# Autodesk Inventor assembly: SpMax_steer
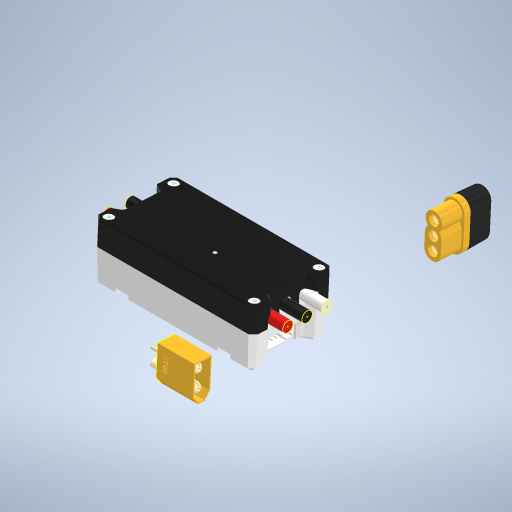
[picture p0: Inventor's stored thumbnail of the model, 512x512]
Saved by Autodesk Inventor 2023 (Build 270158000, 158)
## iProperties
Created: 2023-09-18
Part Number: SpMax_steer
Document SubType Name: Assembly
Designer: shpctac10011
Author: shpctac10011
## Documents named in this file (4)
- G:\.shortcut-targets-by-id\104lhnwPhYvankLacu8RGROV89Bx_24Mg\1939\2_Design\2023-2024\Parts\Electronics\SpMax_steer.iam
- G:\.shortcut-targets-by-id\104lhnwPhYvankLacu8RGROV89Bx_24Mg\1939\2_Design\2023-2024\Parts\Electronics\REV-11-2158-Spark-MAX_Wired.ipt
- G:\.shortcut-targets-by-id\104lhnwPhYvankLacu8RGROV89Bx_24Mg\1939\2_Design\2023-2024\Parts\Electronics\Connectors\XT60_Recp.ipt
- G:\.shortcut-targets-by-id\104lhnwPhYvankLacu8RGROV89Bx_24Mg\1939\2_Design\2023-2024\Parts\Electronics\Connectors\MR60_Plug.iam
## Components (3 placed, 3 different names)
1. REV-11-2158-Spark-MAX_Wired:1 — Flush:1, Flush:2, Flush:3, Mate:1, Mate:2, Mate:3
2. XT60_Recp:1 — Flush:1, Flush:2, Flush:3
3. MR60_Plug:1 [sub-assembly] — Mate:1, Mate:2, Mate:3
## Relationships (6: Flush 3, Mate 3)
- Flush:1 (-25.4 mm): REV-11-2158-Spark-MAX_Wired:1 ↔ XT60_Recp:1
- Flush:2: REV-11-2158-Spark-MAX_Wired:1 ↔ XT60_Recp:1
- Flush:3: REV-11-2158-Spark-MAX_Wired:1 ↔ XT60_Recp:1
- Mate:1 (12.7 mm): REV-11-2158-Spark-MAX_Wired:1 ↔ MR60_Plug:1
- Mate:2 (25.4 mm): REV-11-2158-Spark-MAX_Wired:1 ↔ MR60_Plug:1
- Mate:3 (25.4 mm): REV-11-2158-Spark-MAX_Wired:1 ↔ MR60_Plug:1
